# Autodesk Inventor assembly: Base_3
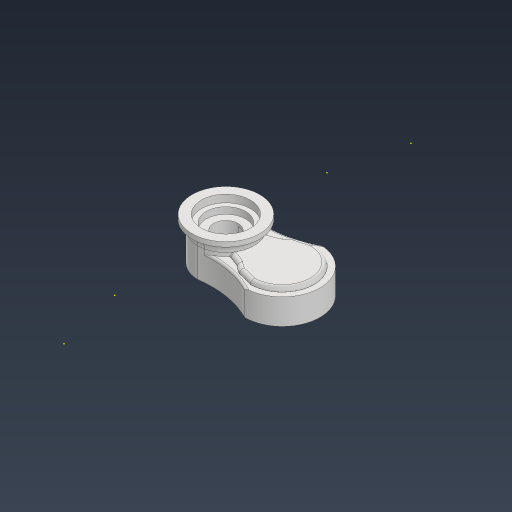
[picture p0: Inventor's stored thumbnail of the model, 512x512]
Saved by Autodesk Inventor 2024 (Build 280153000, 153)
## iProperties
Created: 2025-09-22
Part Number: Base_3
Document SubType Name: Assembly
Designer: Piter
Author: Piter
## Documents named in this file (3)
- C:\Users\Piter\OneDrive\Pulpit\Robots\david_Arm\Davie-Robot-Arm\3D Models\Base_3.iam
- C:\Users\Piter\OneDrive\Pulpit\Robots\david_Arm\Davie-Robot-Arm\3D Models\Base_v3_test.ipt
- C:\Users\Piter\OneDrive\Pulpit\Robots\david_Arm\Davie-Robot-Arm\3D Models\Cover_v2.ipt
## Components (2 placed, 2 different names)
1. Base_v3_test:1 — Flush:1
2. Cover_v2:1 — Flush:1
## Relationships (1: Flush 1)
- Flush:1: Base_v3_test:1 ↔ Cover_v2:1
